# Autodesk Inventor assembly: Head
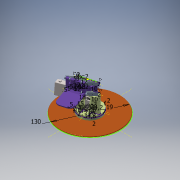
[picture p0: Inventor's stored thumbnail of the model, 180x180]
Saved by Autodesk Inventor 2018.3 (Build 223284000, 284)
## iProperties
Created: 2018-05-16
Part Number: Head
Material: Generisch
Document SubType Name: Assembly
Designer: JochenAlt
Author: JochenAlt
## Documents named in this file (9)
- D:\Projects\Donna\CAD\Head.iam
- D:\Projects\Donna\CAD\Stewart-Head.ipt
- D:\Projects\Donna\CAD\Mouth-Base.ipt
- D:\Projects\Donna\CAD\Servo-KST-DS215MG.ipt
- D:\Projects\Donna\CAD\Rillenkugellager 61707-2RS1.iam
- D:\Projects\Donna\CAD\Mouth-Height-Lever.ipt
- D:\Projects\Donna\CAD\Bottom-Lip.ipt
- D:\Projects\Donna\CAD\Mouth-Height-Lever-front.ipt
- D:\Projects\Donna\CAD\Ball-Joint-male.ipt
## Components (15 placed, 7 different names)
1. Stewart-Plate-Head:1 — Passend:1, Passend:2, Passend:3, Passend:6, Passend:7, Passend:18, Passend:19, Passend:20, Passend:21, Passend:22, Passend:23, Passend:24, Passend:25, Passend:26, Passend:27, Passend:28, Passend:29
2. Mouth-Base:1 — Passend:1, Passend:2, Passend:4, Passend:8, Passend:9, Passend:10, Passend:11, Passend:12
3. Servo-KST-DS215MG:1 — Passend:3, Passend:4, Passend:8
4. Rillenkugellager 61707-2RS1:1 [sub-assembly] — Passend:6, Passend:7
5. Mouth-Height-Lever:1 — Passend:9, Passend:10, Passend:13, Passend:14
6. Bottom-Lip:1 — Passend:11, Passend:12, Passend:15
7. Bottom-Lip:2 — Passend:13, Passend:14, Passend:16, Passend:17
8. Mouth-Height-Lever:2 — Passend:15, Passend:16, Passend:17
9. ball joint:1 — Passend:18, Passend:29
10. ball joint:2 — Passend:19, Passend:28
11. ball joint:3 — Passend:23, Passend:25
12. ball joint:4 — Passend:22, Passend:24
13. ball joint:5 — Passend:21, Passend:27
14. ball joint:6 — Passend:20, Passend:26
15. Servo-KST-DS215MG:2
## Relationships (28: Mate 28)
- Passend:1 [Mate]: Stewart-Plate-Head:1 ↔ Mouth-Base:1
- Passend:2 [Mate] (5 mm): Stewart-Plate-Head:1 ↔ Mouth-Base:1
- Passend:3 [Mate]: Stewart-Plate-Head:1 ↔ Servo-KST-DS215MG:1
- Passend:4 [Mate]: Mouth-Base:1 ↔ Servo-KST-DS215MG:1
- Passend:6 [Mate]: Stewart-Plate-Head:1 ↔ Rillenkugellager 61707-2RS1:1
- Passend:7 [Mate]: Stewart-Plate-Head:1 ↔ Rillenkugellager 61707-2RS1:1
- Passend:8 [Mate]: Mouth-Base:1 ↔ Servo-KST-DS215MG:1
- Passend:9 [Mate]: Mouth-Base:1 ↔ Mouth-Height-Lever:1
- Passend:10 [Mate] (0.5 mm): Mouth-Base:1 ↔ Mouth-Height-Lever:1
- Passend:11 [Mate]: Mouth-Base:1 ↔ Bottom-Lip:1
- Passend:12 [Mate] (0.5 mm): Mouth-Base:1 ↔ Bottom-Lip:1
- Passend:13 [Mate]: Mouth-Height-Lever:1 ↔ Bottom-Lip:2
- Passend:14 [Mate] (0.5 mm): Mouth-Height-Lever:1 ↔ Bottom-Lip:2
- Passend:15 [Mate]: Bottom-Lip:1 ↔ Mouth-Height-Lever:2
- Passend:16 [Mate]: Bottom-Lip:2 ↔ Mouth-Height-Lever:2
- Passend:17 [Mate] (0.5 mm): Bottom-Lip:2 ↔ Mouth-Height-Lever:2
- Passend:18 [Mate]: Stewart-Plate-Head:1 ↔ ball joint:1
- Passend:19 [Mate]: Stewart-Plate-Head:1 ↔ ball joint:2
- Passend:20 [Mate]: Stewart-Plate-Head:1 ↔ ball joint:6
- Passend:21 [Mate]: Stewart-Plate-Head:1 ↔ ball joint:5
- Passend:22 [Mate]: Stewart-Plate-Head:1 ↔ ball joint:4
- Passend:23 [Mate]: Stewart-Plate-Head:1 ↔ ball joint:3
- Passend:24 [Mate]: Stewart-Plate-Head:1 ↔ ball joint:4
- Passend:25 [Mate]: Stewart-Plate-Head:1 ↔ ball joint:3
- Passend:26 [Mate]: Stewart-Plate-Head:1 ↔ ball joint:6
- Passend:27 [Mate]: Stewart-Plate-Head:1 ↔ ball joint:5
- Passend:28 [Mate]: Stewart-Plate-Head:1 ↔ ball joint:2
- Passend:29 [Mate]: Stewart-Plate-Head:1 ↔ ball joint:1
